# Autodesk Inventor assembly: 217-2859-STEP
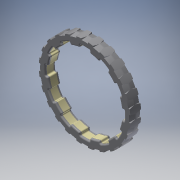
[picture p0: Inventor's stored thumbnail of the model, 180x180]
Saved by Autodesk Inventor 2016 SP2 (Build 200236200, 236)
## iProperties
Created: 2013-12-10
Part Number: 217-2859-STEP
Description: STEP AP214
Document SubType Name: Assembly
Designer: smiku
Mass: 39.854 g
Surface Area: 242.069 cm^2
Volume: 32.2803 cm^3
Density: 1.23462 g/cm^3
Title: 217-2859-STEP.STEP
Revision Number: ANY
Sending System: SolidWorks 2013
Preprocessor: SwSTEP 2.0
## Documents named in this file (3)
- C:\Users\smiku\Downloads\217-2859-2-STEP\217-2859-STEP.iam
- C:\Users\smiku\Downloads\217-2859-2-STEP\217-2859-001 Rev4.ipt
- C:\Users\smiku\Downloads\217-2859-2-STEP\217-2859-011 rev3.ipt
## Components (2 placed, 2 different names)
1. 217-2859-001 Rev4_1 — Rigid:1
2. 217-2859-011 rev3_2 — Rigid:1
## Relationships (1: WeldJoint 1)
- Rigid:1 [WeldJoint]: 217-2859-001 Rev4_1 ↔ 217-2859-011 rev3_2
